# Autodesk Inventor assembly: platform version 2
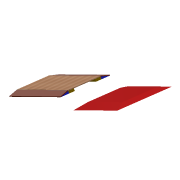
[picture p0: Inventor's stored thumbnail of the model, 180x180]
Saved by Autodesk Inventor 2015 (Build 190159000, 159)
## iProperties
Created: 2015-01-03
Part Number: platform version 2
Document SubType Name: Assembly
Designer: Peter
Mass: 10587 g
Surface Area: 19021.5 cm^2
Volume: 16103.8 cm^3
Density: 0.657427 g/cm^3
Author: Peter
## Documents named in this file (9)
- T:\FILES\FIRST-Team-1719-CAD-Team\2015 Playing Field\Team 1719 Practice Field\Scoring Platform - Construction Design\platform version 2.iam
- T:\FILES\FIRST-Team-1719-CAD-Team\2015 Playing Field\Team 1719 Practice Field\Scoring Platform - Construction Design\plywood platform.ipt
- T:\FILES\FIRST-Team-1719-CAD-Team\2015 Playing Field\Team 1719 Practice Field\Scoring Platform - Construction Design\2x4x48.ipt
- T:\FILES\FIRST-Team-1719-CAD-Team\2015 Playing Field\Team 1719 Practice Field\Scoring Platform - Construction Design\loft version.ipt
- T:\FILES\FIRST-Team-1719-CAD-Team\2015 Playing Field\Team 1719 Practice Field\Scoring Platform - Construction Design\Ramp Assembly Version 2.iam
- T:\FILES\FIRST-Team-1719-CAD-Team\2015 Playing Field\Team 1719 Practice Field\Scoring Platform - Construction Design\Wedge version 2.ipt
- T:\FILES\FIRST-Team-1719-CAD-Team\2015 Playing Field\Team 1719 Practice Field\Scoring Platform - Construction Design\2x4x48_MIR.ipt
- T:\FILES\FIRST-Team-1719-CAD-Team\2015 Playing Field\Team 1719 Practice Field\Scoring Platform - Construction Design\Wedge version 2_MIR.ipt
- T:\FILES\FIRST-Team-1719-CAD-Team\2015 Playing Field\Team 1719 Practice Field\Scoring Platform - Construction Design\Ramp Assembly Version 2_MIR.iam
## Components (15 placed, 8 different names)
1. plywood platform:1 — Mate:1, Flush:1, Flush:2, Flush:3, Flush:4, Mate:2, Rotational:1
2. 2x4x48:1 — Mate:1, Flush:1, Flush:2
3. 2x4x48:2 — Flush:3, Flush:4, Mate:2, Mate:3, Mate:4, Mate:5, Mate:6, Flush:5, Flush:6, Flush:7, Flush:8, Flush:9, Flush:10
4. loft version:1
5. Ramp Assembly Version 2:1 [sub-assembly] — Rotational:1, Mate:15
6. Wedge version 2:1 — Mate:3, Flush:5, Flush:10, Mate:7
7. Wedge version 2:2 — Mate:6, Flush:6, Mate:7
8. Wedge version 2:3 — Mate:5, Flush:7, Mate:8
9. Wedge version 2:4 — Mate:4, Flush:8, Flush:9, Mate:8, Mate:15
10. 2x4x48_MIR:1 — Flush:11, Flush:12, Mate:9, Flush:13, Mate:11, Flush:14, Mate:12, Flush:15, Flush:16, Mate:14
11. Wedge version 2_MIR:1 — Flush:11, Flush:12, Mate:9, Mate:10
12. Wedge version 2_MIR:2 — Mate:10, Flush:13, Mate:11
13. Wedge version 2_MIR:3 — Flush:14, Mate:12, Mate:13
14. Wedge version 2_MIR:4 — Mate:13, Flush:15, Flush:16, Mate:14
15. Ramp Assembly Version 2_MIR:1 [sub-assembly]
## Relationships (32: Flush 16, Mate 15, RevoluteJoint 1)
- Mate:1: plywood platform:1 ↔ 2x4x48:1
- Flush:1: plywood platform:1 ↔ 2x4x48:1
- Flush:2: plywood platform:1 ↔ 2x4x48:1
- Flush:3: plywood platform:1 ↔ 2x4x48:2
- Flush:4: plywood platform:1 ↔ 2x4x48:2
- Mate:2: plywood platform:1 ↔ 2x4x48:2
- Rotational:1 [RevoluteJoint]: plywood platform:1 ↔ Ramp Assembly Version 2:1
- Mate:3: 2x4x48:2 ↔ Wedge version 2:1
- Mate:4: 2x4x48:2 ↔ Wedge version 2:4
- Mate:5: 2x4x48:2 ↔ Wedge version 2:3
- Mate:6: 2x4x48:2 ↔ Wedge version 2:2
- Flush:5: 2x4x48:2 ↔ Wedge version 2:1
- Flush:6: 2x4x48:2 ↔ Wedge version 2:2
- Flush:7: 2x4x48:2 ↔ Wedge version 2:3
- Flush:8: 2x4x48:2 ↔ Wedge version 2:4
- Flush:9: 2x4x48:2 ↔ Wedge version 2:4
- Flush:10: 2x4x48:2 ↔ Wedge version 2:1
- Mate:7 (491.0667 mm): Wedge version 2:1 ↔ Wedge version 2:2
- Mate:8 (491.0667 mm): Wedge version 2:3 ↔ Wedge version 2:4
- Flush:11: 2x4x48_MIR:1 ↔ Wedge version 2_MIR:1
- Flush:12: 2x4x48_MIR:1 ↔ Wedge version 2_MIR:1
- Mate:9: 2x4x48_MIR:1 ↔ Wedge version 2_MIR:1
- Mate:10 (491.0667 mm): Wedge version 2_MIR:1 ↔ Wedge version 2_MIR:2
- Flush:13: 2x4x48_MIR:1 ↔ Wedge version 2_MIR:2
- Mate:11: 2x4x48_MIR:1 ↔ Wedge version 2_MIR:2
- Flush:14: 2x4x48_MIR:1 ↔ Wedge version 2_MIR:3
- Mate:12: 2x4x48_MIR:1 ↔ Wedge version 2_MIR:3
- Mate:13 (491.0667 mm): Wedge version 2_MIR:3 ↔ Wedge version 2_MIR:4
- Flush:15: 2x4x48_MIR:1 ↔ Wedge version 2_MIR:4
- Flush:16: 2x4x48_MIR:1 ↔ Wedge version 2_MIR:4
- Mate:14: 2x4x48_MIR:1 ↔ Wedge version 2_MIR:4
- Mate:15: Ramp Assembly Version 2:1 ↔ Wedge version 2:4
